# Autodesk Inventor assembly: GE-12019
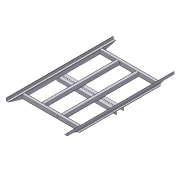
[picture p0: Inventor's stored thumbnail of the model, 180x180]
Saved by Autodesk Inventor 2012 (Build 160160000, 160)
## iProperties
Created: 2011-06-06
Part Number: GE-12019
Document SubType Name: Assembly
Designer: dfoster
Description: Bridge, Frame
Title: Bridge, Frame
Author: dfoster
## Documents named in this file (7)
- C:\Data Folder\FRC 2012 Field\Components\GE-12019.iam
- C:\Data Folder\FRC 2012 Field\Components\GE-12019-01.ipt
- C:\Data Folder\FRC 2012 Field\Components\GE-12019-02.ipt
- C:\Data Folder\FRC 2012 Field\Components\GE-12019-03.ipt
- C:\Data Folder\FRC 2012 Field\Components\GE-12019-05.ipt
- C:\Data Folder\FRC 2012 Field\Components\GE-12019-06.ipt
- C:\Data Folder\FRC 2012 Field\Components\GE-12019-04.ipt
## Components (12 placed, 6 different names)
1. GE-12019-01:1 — Flush:1, Mate:1, Flush:2, Flush:17
2. GE-12019-01:2 — Flush:1, Mate:1, Flush:2, Flush:3, Flush:18
3. GE-12019-02:2 — Mate:4, Flush:11, Mate:6, Flush:19, Flush:26, Flush:27
4. GE-12019-02:4 — Mate:15, Flush:26, Mate:16
5. GE-12019-03:1 — Flush:3, Flush:18, Flush:20, Flush:27, Flush:28
6. GE-12019-03:2 — Mate:4, Flush:11, Mate:9, Mate:10, Flush:16, Flush:17, Mate:15, Flush:28
7. GE-12019-06:1 — Mate:10, Flush:16, Mate:11, Flush:20, Flush:21, Flush:22, Flush:23, Mate:13, Mate:14
8. GE-12019-06:2 — Mate:9, Mate:11, Flush:21
9. GE-12019-04:1 — Flush:22, Flush:25, Mate:13
10. GE-12019-04:2 — Flush:23, Flush:24, Mate:14
11. GE-12019-05:1 — Mate:6, Flush:19, Flush:24
12. GE-12019-05:2 — Flush:25, Mate:16
## Component patterns: (2 elements, first: GE-12019-05:1)
## Relationships (30: Flush 17, Mate 13)
- Flush:1: GE-12019-01:1 ↔ GE-12019-01:2
- Mate:1 (-1219.2 mm): GE-12019-01:1 ↔ GE-12019-01:2
- Flush:2: GE-12019-01:1 ↔ GE-12019-01:2
- Flush:3 (25.4 mm): GE-12019-01:2 ↔ GE-12019-03:1
- [Mate]: GE-12019-01:2 ↔ GE-12019-03:1
- [Mate]: GE-12019-01:1 ↔ GE-12019-03:2
- [Mate] (336.55 mm): GE-12019-03:1 ↔ GE-12019-05:1
- Mate:4: GE-12019-02:2 ↔ GE-12019-03:2
- Flush:11 (6.35 mm): GE-12019-02:2 ↔ GE-12019-03:2
- Mate:6: GE-12019-02:2 ↔ GE-12019-05:1
- Mate:9: GE-12019-03:2 ↔ GE-12019-06:2
- Mate:10: GE-12019-03:2 ↔ GE-12019-06:1
- Flush:16 (968.375 mm): GE-12019-03:2 ↔ GE-12019-06:1
- Mate:11 (-146.05 mm): GE-12019-06:1 ↔ GE-12019-06:2
- Flush:17: GE-12019-01:1 ↔ GE-12019-03:2
- Flush:18: GE-12019-01:2 ↔ GE-12019-03:1
- Flush:19: GE-12019-02:2 ↔ GE-12019-05:1
- Flush:20 (6.35 mm): GE-12019-03:1 ↔ GE-12019-06:1
- Flush:21: GE-12019-06:1 ↔ GE-12019-06:2
- Flush:22: GE-12019-06:1 ↔ GE-12019-04:1
- Flush:23: GE-12019-06:1 ↔ GE-12019-04:2
- Flush:24: GE-12019-04:2 ↔ GE-12019-05:1
- Flush:25: GE-12019-04:1 ↔ GE-12019-05:2
- Mate:13: GE-12019-06:1 ↔ GE-12019-04:1
- Mate:14: GE-12019-06:1 ↔ GE-12019-04:2
- Mate:15: GE-12019-02:4 ↔ GE-12019-03:2
- Flush:26: GE-12019-02:2 ↔ GE-12019-02:4
- Mate:16: GE-12019-02:4 ↔ GE-12019-05:2
- Flush:27 (241.3 mm): GE-12019-02:2 ↔ GE-12019-03:1
- Flush:28: GE-12019-03:1 ↔ GE-12019-03:2
